# Autodesk Inventor assembly: Motor-Assy
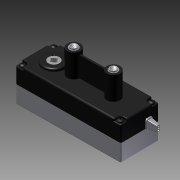
[picture p0: Inventor's stored thumbnail of the model, 180x180]
Saved by Autodesk Inventor 2013 (Build 170138000, 138)
## iProperties
Created: 2011-03-18
Part Number: Motor-Assy
Document SubType Name: Assembly
Designer: vex_intern
Author: vex_intern
## Documents named in this file (10)
- C:\Data Folder\VEX 2012\VEX KOP Uploads\2013\Metric\Motion\Components\Motor-Assy.iam
- C:\Data Folder\VEX 2012\VEX KOP Uploads\2013\Metric\Motion\Components\E535-SERVO-BEARING-A_1.ipt
- C:\Data Folder\VEX 2012\VEX KOP Uploads\2013\Metric\Motion\Components\EXISTING-WIRE-SUPPORT_1.ipt
- C:\Data Folder\VEX 2012\VEX KOP Uploads\2013\Metric\Motion\Components\TZ2_1.ipt
- C:\Data Folder\VEX 2012\VEX KOP Uploads\2013\Metric\Motion\Components\BOTTOM_1.ipt
- C:\Data Folder\VEX 2012\VEX KOP Uploads\2013\Metric\Motion\Components\B-M7Z28_1.ipt
- C:\Data Folder\VEX 2012\VEX KOP Uploads\2013\Metric\Motion\Components\TOP_1.ipt
- C:\Data Folder\VEX 2012\VEX KOP Uploads\2013\Metric\Motion\Components\RING_1.ipt
- C:\Data Folder\VEX 2012\VEX KOP Uploads\2013\Metric\Motion\Components\E535-SERVO-NUT_1.ipt
- C:\Data Folder\VEX 2012\VEX KOP Uploads\2013\Metric\Motion\Components\ANSI B18.6.3 - 1-64 UNC - 0.1875(4A).ipt
## Components (13 placed, 9 different names)
1. E535-SERVO-BEARING-A_1:1 — Insert:8
2. EXISTING-WIRE-SUPPORT_1:1 — Mate:6, Mate:7, Mate:8
3. TZ2_1:1 — Insert:9
4. BOTTOM_1:1 — Insert:1, Insert:2, Insert:3, Insert:4, Mate:5, Flush:1, Insert:5, Insert:6, Mate:6, Mate:7, Mate:8, Mate:9, Mate:10, Mate:11, Insert:7, Insert:8
5. B-M7Z28_1:1 — Mate:1, Angle:1, Mate:2, Angle:2, Mate:5, Flush:1
6. TOP_1:1 — Mate:9, Mate:10, Mate:11
7. RING_1:1 — Insert:7, Insert:9
8. E535-SERVO-NUT_1:1 — Insert:5
9. E535-SERVO-NUT_1:2 — Insert:6
10. Cross Recessed Pan Head Machine Screw - Type I - Inch No. 1 - 64 - 3/16:1 — Insert:1
11. Cross Recessed Pan Head Machine Screw - Type I - Inch No. 1 - 64 - 3/16:2 — Insert:4
12. Cross Recessed Pan Head Machine Screw - Type I - Inch No. 1 - 64 - 3/16:3 — Insert:3
13. Cross Recessed Pan Head Machine Screw - Type I - Inch No. 1 - 64 - 3/16:4 — Insert:2
## Relationships (23: Mate 11, Insert 9, Angle 2, Flush 1)
- Insert:1: BOTTOM_1:1 ↔ Cross Recessed Pan Head Machine Screw - Type I - Inch No. 1 - 64 - 3/16:1
- Insert:2: BOTTOM_1:1 ↔ Cross Recessed Pan Head Machine Screw - Type I - Inch No. 1 - 64 - 3/16:4
- Insert:3: BOTTOM_1:1 ↔ Cross Recessed Pan Head Machine Screw - Type I - Inch No. 1 - 64 - 3/16:3
- Insert:4: BOTTOM_1:1 ↔ Cross Recessed Pan Head Machine Screw - Type I - Inch No. 1 - 64 - 3/16:2
- Mate:1: B-M7Z28_1:1
- Angle:1 (0 deg): B-M7Z28_1:1
- Mate:2: B-M7Z28_1:1
- Angle:2 (0 deg): B-M7Z28_1:1
- Mate:3
- Mate:4
- Mate:5: BOTTOM_1:1 ↔ B-M7Z28_1:1
- Flush:1: BOTTOM_1:1 ↔ B-M7Z28_1:1
- Insert:5: BOTTOM_1:1 ↔ E535-SERVO-NUT_1:1
- Insert:6: BOTTOM_1:1 ↔ E535-SERVO-NUT_1:2
- Mate:6: EXISTING-WIRE-SUPPORT_1:1 ↔ BOTTOM_1:1
- Mate:7: EXISTING-WIRE-SUPPORT_1:1 ↔ BOTTOM_1:1
- Mate:8: EXISTING-WIRE-SUPPORT_1:1 ↔ BOTTOM_1:1
- Mate:9: BOTTOM_1:1 ↔ TOP_1:1
- Mate:10: BOTTOM_1:1 ↔ TOP_1:1
- Mate:11: BOTTOM_1:1 ↔ TOP_1:1
- Insert:7: BOTTOM_1:1 ↔ RING_1:1
- Insert:8: E535-SERVO-BEARING-A_1:1 ↔ BOTTOM_1:1
- Insert:9: TZ2_1:1 ↔ RING_1:1
